# Autodesk Inventor assembly: CuboidSecurityBox
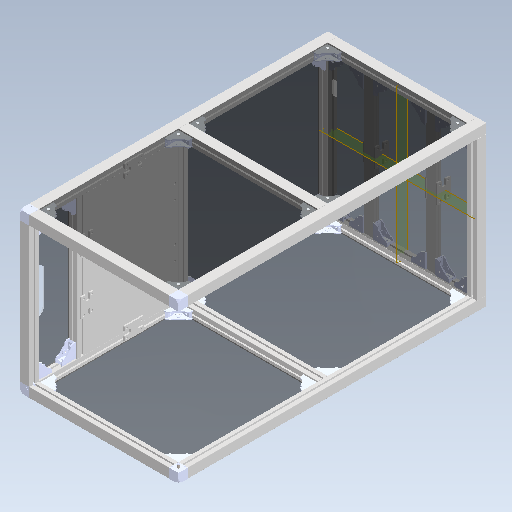
[picture p0: Inventor's stored thumbnail of the model, 512x512]
Saved by Autodesk Inventor 2021 (Build 250183000, 183)
## iProperties
Created: 2020-11-05
Part Number: CuboidSecurityBox
Document SubType Name: Assembly
Designer: gisen
Author: gisen
## Documents named in this file (12)
- D:\GitProjects\CAD-Data\CuboidAccessories\SecurityBox\Assemblies\CuboidSecurityBoxBasis.iam
- D:\GitProjects\CAD-Data\CuboidAccessories\SecurityBox\Frames\BasicFrameSingleSide290.ipt
- D:\GitProjects\CAD-Data\GeneralComponentsTemplate\Fittings\BasicFrameBracket.ipt
- D:\GitProjects\CAD-Data\CuboidAccessories\SecurityBox\Frames\BasicFrameCornerSide620.ipt
- D:\GitProjects\CAD-Data\CuboidAccessories\SecurityBox\Frames\BasicFrameLight290.ipt
- D:\GitProjects\CAD-Data\CuboidAccessories\SecurityBox\Misc\HTypeMount.ipt
- D:\GitProjects\CAD-Data\GeneralComponentsTemplate\Fittings\BasicFrameCubeBracket.iam
- D:\GitProjects\CAD-Data\CuboidAccessories\SecurityBox\Plates\InsideBottomPlate.ipt
- D:\GitProjects\CAD-Data\CuboidAccessories\SecurityBox\Assemblies\iPadHolderAssembly.iam
- D:\GitProjects\CAD-Data\CuboidAccessories\SecurityBox\Frames\BasicFrameCornerSide290.ipt
- D:\GitProjects\CAD-Data\CuboidAccessories\SecurityBox\Plates\OutsideSidePlate.ipt
- D:\GitProjects\CAD-Data\CuboidAccessories\SecurityBox\Plates\OutsideBackSideHigherPlate.ipt
## Components (73 placed, 11 different names)
1. BasicFrameSingleSide290:1 — フラッシュ:3, メイト:38, メイト:39, フラッシュ:21, フラッシュ:23, メイト:41, メイト:52, メイト:60, メイト:62, メイト:64, メイト:65, メイト:129, メイト:177, メイト:224, 対称度:1
2. BasicFrameSingleSide290:2 — フラッシュ:22, フラッシュ:24, フラッシュ:25, フラッシュ:26, メイト:40, メイト:42, メイト:43, メイト:44, メイト:45, メイト:104, メイト:107, メイト:110, メイト:113, フラッシュ:43, メイト:128, 対称度:2, メイト:239, メイト:241
3. BasicFrameSingleSide290:3 — フラッシュ:15, フラッシュ:18, メイト:35, フラッシュ:27, メイト:46, メイト:47, メイト:50, メイト:55, メイト:67, メイト:68, メイト:69, メイト:71, メイト:214, メイト:218, 対称度:1
4. BasicFrameSingleSide290:4 — フラッシュ:3, フラッシュ:16, フラッシュ:17, メイト:36, フラッシュ:19, メイト:37, フラッシュ:20, メイト:48, メイト:49, メイト:51, メイト:53, メイト:54, メイト:56, メイト:57, メイト:59, フラッシュ:32, フラッシュ:33, メイト:92, メイト:95, メイト:98, メイト:101, 対称度:2
5. BasicFrameBracket:23 — メイト:48, メイト:49, メイト:50
6. BasicFrameBracket:27 — メイト:45, メイト:46, メイト:47
7. BasicFrameBracket:28 — メイト:51, メイト:52, メイト:53
8. BasicFrameCornerSide620:1 — フラッシュ:25, フラッシュ:26, メイト:40, フラッシュ:27, メイト:66, メイト:126, フラッシュ:39, フラッシュ:40, メイト:158, メイト:157, メイト:183, メイト:203, メイト:204, メイト:215
9. BasicFrameCornerSide620:2 — メイト:39, フラッシュ:21, フラッシュ:22, フラッシュ:23, フラッシュ:24, メイト:43, メイト:63, メイト:127, フラッシュ:41, フラッシュ:42, メイト:167, メイト:168, メイト:169, メイト:191, フラッシュ:80, メイト:199, メイト:201, メイト:223
10. BasicFrameCornerSide620:3 — フラッシュ:19, メイト:37, フラッシュ:20, メイト:38, メイト:58, メイト:61, メイト:135, フラッシュ:47, メイト:147, フラッシュ:52, フラッシュ:53, メイト:163, メイト:165, フラッシュ:61, メイト:187, メイト:197, メイト:198, メイト:211, メイト:213, メイト:220, メイト:222
11. BasicFrameCornerSide620:4 — フラッシュ:15, フラッシュ:16, フラッシュ:17, フラッシュ:18, メイト:35, メイト:36, メイト:70, メイト:148, フラッシュ:54, フラッシュ:55, メイト:154, メイト:159, メイト:161, メイト:172, フラッシュ:63, メイト:186, メイト:205, メイト:207, メイト:209, メイト:210, メイト:217, メイト:226
12. BasicFrameBracket:29 — メイト:41, メイト:42, メイト:44
13. BasicFrameBracket:30 — メイト:54, メイト:55, メイト:56
14. BasicFrameBracket:31 — メイト:57, メイト:58, メイト:59
15. BasicFrameBracket:33 — メイト:66, メイト:67, メイト:68
16. BasicFrameBracket:34 — メイト:69, メイト:70, メイト:71
17. BasicFrameBracket:35 — メイト:63, メイト:64, メイト:65
18. BasicFrameBracket:37 — メイト:60, メイト:61, メイト:62
19. BasicFrameLight290:1 — フラッシュ:32, メイト:88, メイト:91, メイト:93, メイト:102, メイト:106, メイト:120, メイト:121, メイト:122, メイト:123, メイト:124, メイト:125, フラッシュ:64, フラッシュ:65, フラッシュ:66, フラッシュ:67, フラッシュ:68, メイト:177
20. BasicFrameLight290:2 — フラッシュ:33, メイト:88, メイト:97, メイト:99, メイト:108, メイト:112, メイト:114, メイト:115, メイト:116, メイト:117, メイト:118, メイト:119, フラッシュ:68, フラッシュ:69, フラッシュ:70, フラッシュ:71, フラッシュ:72, フラッシュ:73, メイト:241
21. BasicFrameBracket:38 — メイト:91, メイト:92, フラッシュ:64
22. BasicFrameBracket:39 — メイト:93, メイト:95, フラッシュ:65
23. BasicFrameBracket:40 — メイト:102, メイト:104, フラッシュ:66
24. BasicFrameBracket:41 — メイト:106, メイト:107, フラッシュ:67
25. BasicFrameBracket:42 — メイト:97, メイト:98, フラッシュ:69
26. BasicFrameBracket:43 — メイト:99, メイト:101, フラッシュ:70
27. BasicFrameBracket:44 — メイト:108, メイト:110, フラッシュ:71
28. BasicFrameBracket:45 — メイト:112, メイト:113, フラッシュ:72
29. HTypeMount:1 — メイト:114, メイト:115, メイト:116, フラッシュ:35
30. HTypeMount:2 — メイト:117, メイト:118, メイト:119, フラッシュ:35, フラッシュ:37, フラッシュ:73
31. HTypeMount:3 — メイト:123, メイト:124, メイト:125, フラッシュ:36, フラッシュ:37
32. HTypeMount:4 — メイト:120, メイト:121, メイト:122, フラッシュ:36
33. BasicFrameCubeBracket:1 [sub-assembly] — メイト:126, フラッシュ:39, フラッシュ:40, フラッシュ:76
34. BasicFrameCubeBracket:2 [sub-assembly] — メイト:127, フラッシュ:41, フラッシュ:42, メイト:195
35. InsideBottomPlate:1 — フラッシュ:43, メイト:128, メイト:129
36. BasicFrameSingleSide290:5 — メイト:130, メイト:131, フラッシュ:44, メイト:132, メイト:133, フラッシュ:45, メイト:134, フラッシュ:46, フラッシュ:47, フラッシュ:48, フラッシュ:57, フラッシュ:60, フラッシュ:62, フラッシュ:83, メイト:219
37. BasicFrameBracket:46 — メイト:130, メイト:131, フラッシュ:44, メイト:135
38. BasicFrameBracket:47 — メイト:132, メイト:133, フラッシュ:45
39. BasicFrameSingleSide290:6 — メイト:134, フラッシュ:46, フラッシュ:48, メイト:137, メイト:138, メイト:139, メイト:140, フラッシュ:50, フラッシュ:51, メイト:153, フラッシュ:88, メイト:225
40. BasicFrameBracket:48 — メイト:139, メイト:140, フラッシュ:50
41. BasicFrameBracket:49 — メイト:137, メイト:138, フラッシュ:51
42. BasicFrameCubeBracket:3 [sub-assembly] — メイト:147, フラッシュ:52, フラッシュ:53, メイト:194
43. BasicFrameCubeBracket:4 [sub-assembly] — メイト:148, フラッシュ:54, フラッシュ:55, メイト:193, フラッシュ:75, フラッシュ:77, フラッシュ:78
44. iPadHolderAssembly:1 [sub-assembly] — メイト:153, フラッシュ:57, メイト:154, メイト:227, メイト:228, メイト:229, メイト:230, メイト:231, メイト:232, メイト:233, メイト:234, メイト:235, メイト:236, メイト:237, メイト:238
45. BasicFrameBracket:52 — メイト:157, メイト:158, メイト:174
46. BasicFrameBracket:53 — メイト:163, メイト:165, メイト:171
47. BasicFrameBracket:54 — メイト:159, メイト:161, メイト:173
48. BasicFrameBracket:55 — メイト:167, メイト:168, メイト:170
49. BasicFrameSingleSide290:7 — メイト:169, メイト:170, フラッシュ:60, メイト:171, フラッシュ:61, メイト:188, メイト:189, メイト:190, メイト:192, フラッシュ:84, フラッシュ:85
50. BasicFrameSingleSide290:8 — メイト:172, フラッシュ:62, フラッシュ:63, メイト:173, メイト:174, メイト:181, メイト:182, メイト:184, メイト:185, メイト:214, フラッシュ:82
51. BasicFrameBracket:56 — メイト:181, メイト:182, メイト:183
52. BasicFrameBracket:57 — メイト:184, メイト:185, メイト:186
53. BasicFrameBracket:58 — メイト:187, メイト:188, メイト:189
54. BasicFrameBracket:59 — メイト:190, メイト:191, メイト:192
55. BasicFrameCornerSide290:1 — メイト:193, フラッシュ:75, フラッシュ:76, メイト:202, メイト:206, フラッシュ:81, メイト:216
56. BasicFrameCornerSide290:3 — メイト:194, フラッシュ:77, フラッシュ:78, フラッシュ:79, メイト:208, メイト:212
57. BasicFrameCornerSide290:4 — メイト:195, フラッシュ:79, フラッシュ:80, メイト:196, メイト:200, メイト:221
58. BasicFrameBracket:60 — メイト:196, メイト:197, メイト:198
59. BasicFrameBracket:61 — メイト:199, メイト:200, メイト:201
60. BasicFrameBracket:62 — メイト:202, メイト:203, メイト:204
61. BasicFrameBracket:63 — メイト:205, メイト:206, メイト:207
62. BasicFrameBracket:64 — メイト:211, メイト:212, メイト:213
63. BasicFrameBracket:65 — メイト:208, メイト:209, メイト:210
64. OutsideSidePlate:1 — フラッシュ:83, メイト:219, メイト:220
65. OutsideSidePlate:2 — フラッシュ:82, メイト:217, メイト:218
66. OutsideSidePlate:3 — フラッシュ:81, メイト:215, メイト:216
67. OutsideSidePlate:4 — フラッシュ:85, メイト:223, メイト:224
68. OutsideSidePlate:5 — フラッシュ:84, メイト:221, メイト:222
69. OutsideBackSideHigherPlate:1 — フラッシュ:88, メイト:225, メイト:226
70. HTypeMount:5 — メイト:236, メイト:237, メイト:238
71. HTypeMount:6 — メイト:233, メイト:234, メイト:235
72. HTypeMount:7 — メイト:227, メイト:228, メイト:229
73. HTypeMount:8 — メイト:230, メイト:231, メイト:232
## Relationships (225: Mate 161, Flush 62, Symmetry 2)
- フラッシュ:3 [Flush]: BasicFrameSingleSide290:1 ↔ BasicFrameSingleSide290:4
- フラッシュ:15 [Flush]: BasicFrameSingleSide290:3 ↔ BasicFrameCornerSide620:4
- フラッシュ:16 [Flush]: BasicFrameSingleSide290:4 ↔ BasicFrameCornerSide620:4
- フラッシュ:17 [Flush]: BasicFrameSingleSide290:4 ↔ BasicFrameCornerSide620:4
- フラッシュ:18 [Flush]: BasicFrameSingleSide290:3 ↔ BasicFrameCornerSide620:4
- メイト:35 [Mate]: BasicFrameSingleSide290:3 ↔ BasicFrameCornerSide620:4
- メイト:36 [Mate]: BasicFrameSingleSide290:4 ↔ BasicFrameCornerSide620:4
- フラッシュ:19 [Flush]: BasicFrameSingleSide290:4 ↔ BasicFrameCornerSide620:3
- メイト:37 [Mate]: BasicFrameSingleSide290:4 ↔ BasicFrameCornerSide620:3
- フラッシュ:20 [Flush]: BasicFrameSingleSide290:4 ↔ BasicFrameCornerSide620:3
- メイト:38 [Mate]: BasicFrameSingleSide290:1 ↔ BasicFrameCornerSide620:3
- メイト:39 [Mate]: BasicFrameSingleSide290:1 ↔ BasicFrameCornerSide620:2
- フラッシュ:21 [Flush]: BasicFrameSingleSide290:1 ↔ BasicFrameCornerSide620:2
- フラッシュ:22 [Flush]: BasicFrameSingleSide290:2 ↔ BasicFrameCornerSide620:2
- フラッシュ:23 [Flush]: BasicFrameSingleSide290:1 ↔ BasicFrameCornerSide620:2
- フラッシュ:24 [Flush]: BasicFrameSingleSide290:2 ↔ BasicFrameCornerSide620:2
- フラッシュ:25 [Flush]: BasicFrameSingleSide290:2 ↔ BasicFrameCornerSide620:1
- フラッシュ:26 [Flush]: BasicFrameSingleSide290:2 ↔ BasicFrameCornerSide620:1
- メイト:40 [Mate]: BasicFrameSingleSide290:2 ↔ BasicFrameCornerSide620:1
- メイト:41 [Mate]: BasicFrameSingleSide290:1 ↔ BasicFrameBracket:29
- メイト:42 [Mate] (-10 mm): BasicFrameSingleSide290:2 ↔ BasicFrameBracket:29
- メイト:43 [Mate]: BasicFrameSingleSide290:2 ↔ BasicFrameCornerSide620:2
- フラッシュ:27 [Flush]: BasicFrameSingleSide290:3 ↔ BasicFrameCornerSide620:1
- メイト:44 [Mate]: BasicFrameSingleSide290:2 ↔ BasicFrameBracket:29
- メイト:45 [Mate]: BasicFrameSingleSide290:2 ↔ BasicFrameBracket:27
- メイト:46 [Mate]: BasicFrameSingleSide290:3 ↔ BasicFrameBracket:27
- メイト:47 [Mate] (-10 mm): BasicFrameSingleSide290:3 ↔ BasicFrameBracket:27
- メイト:48 [Mate]: BasicFrameSingleSide290:4 ↔ BasicFrameBracket:23
- メイト:49 [Mate] (-10 mm): BasicFrameSingleSide290:4 ↔ BasicFrameBracket:23
- メイト:50 [Mate]: BasicFrameSingleSide290:3 ↔ BasicFrameBracket:23
- メイト:51 [Mate]: BasicFrameSingleSide290:4 ↔ BasicFrameBracket:28
- メイト:52 [Mate]: BasicFrameSingleSide290:1 ↔ BasicFrameBracket:28
- メイト:53 [Mate] (-10 mm): BasicFrameSingleSide290:4 ↔ BasicFrameBracket:28
- メイト:54 [Mate]: BasicFrameSingleSide290:4 ↔ BasicFrameBracket:30
- メイト:55 [Mate]: BasicFrameSingleSide290:3 ↔ BasicFrameBracket:30
- メイト:56 [Mate] (-10 mm): BasicFrameSingleSide290:4 ↔ BasicFrameBracket:30
- メイト:57 [Mate]: BasicFrameSingleSide290:4 ↔ BasicFrameBracket:31
- メイト:58 [Mate]: BasicFrameCornerSide620:3 ↔ BasicFrameBracket:31
- メイト:59 [Mate] (-10 mm): BasicFrameSingleSide290:4 ↔ BasicFrameBracket:31
- メイト:60 [Mate] (-10 mm): BasicFrameSingleSide290:1 ↔ BasicFrameBracket:37
- メイト:61 [Mate]: BasicFrameCornerSide620:3 ↔ BasicFrameBracket:37
- メイト:62 [Mate]: BasicFrameSingleSide290:1 ↔ BasicFrameBracket:37
- メイト:63 [Mate]: BasicFrameCornerSide620:2 ↔ BasicFrameBracket:35
- メイト:64 [Mate]: BasicFrameSingleSide290:1 ↔ BasicFrameBracket:35
- メイト:65 [Mate] (-10 mm): BasicFrameSingleSide290:1 ↔ BasicFrameBracket:35
- メイト:66 [Mate]: BasicFrameCornerSide620:1 ↔ BasicFrameBracket:33
- メイト:67 [Mate]: BasicFrameSingleSide290:3 ↔ BasicFrameBracket:33
- メイト:68 [Mate] (-10 mm): BasicFrameSingleSide290:3 ↔ BasicFrameBracket:33
- メイト:69 [Mate]: BasicFrameSingleSide290:3 ↔ BasicFrameBracket:34
- メイト:70 [Mate]: BasicFrameCornerSide620:4 ↔ BasicFrameBracket:34
- メイト:71 [Mate] (-10 mm): BasicFrameSingleSide290:3 ↔ BasicFrameBracket:34
- フラッシュ:32 [Flush] (5 mm): BasicFrameSingleSide290:4 ↔ BasicFrameLight290:1
- フラッシュ:33 [Flush] (5 mm): BasicFrameSingleSide290:4 ↔ BasicFrameLight290:2
- メイト:88 [Mate] (110 mm): BasicFrameLight290:1 ↔ BasicFrameLight290:2
- メイト:91 [Mate]: BasicFrameLight290:1 ↔ BasicFrameBracket:38
- メイト:92 [Mate] (-10 mm): BasicFrameSingleSide290:4 ↔ BasicFrameBracket:38
- メイト:93 [Mate]: BasicFrameLight290:1 ↔ BasicFrameBracket:39
- メイト:95 [Mate] (-10 mm): BasicFrameSingleSide290:4 ↔ BasicFrameBracket:39
- メイト:97 [Mate]: BasicFrameLight290:2 ↔ BasicFrameBracket:42
- メイト:98 [Mate] (-10 mm): BasicFrameSingleSide290:4 ↔ BasicFrameBracket:42
- メイト:99 [Mate]: BasicFrameLight290:2 ↔ BasicFrameBracket:43
- メイト:101 [Mate] (-10 mm): BasicFrameSingleSide290:4 ↔ BasicFrameBracket:43
- メイト:102 [Mate]: BasicFrameLight290:1 ↔ BasicFrameBracket:40
- メイト:104 [Mate] (-10 mm): BasicFrameSingleSide290:2 ↔ BasicFrameBracket:40
- メイト:106 [Mate]: BasicFrameLight290:1 ↔ BasicFrameBracket:41
- メイト:107 [Mate] (-10 mm): BasicFrameSingleSide290:2 ↔ BasicFrameBracket:41
- メイト:108 [Mate]: BasicFrameLight290:2 ↔ BasicFrameBracket:44
- メイト:110 [Mate] (-10 mm): BasicFrameSingleSide290:2 ↔ BasicFrameBracket:44
- メイト:112 [Mate]: BasicFrameLight290:2 ↔ BasicFrameBracket:45
- メイト:113 [Mate] (-10 mm): BasicFrameSingleSide290:2 ↔ BasicFrameBracket:45
- メイト:114 [Mate]: BasicFrameLight290:2 ↔ HTypeMount:1
- メイト:115 [Mate] (-5 mm): BasicFrameLight290:2 ↔ HTypeMount:1
- メイト:116 [Mate] (-5 mm): BasicFrameLight290:2 ↔ HTypeMount:1
- メイト:117 [Mate]: BasicFrameLight290:2 ↔ HTypeMount:2
- メイト:118 [Mate] (-5 mm): BasicFrameLight290:2 ↔ HTypeMount:2
- メイト:119 [Mate] (-5 mm): BasicFrameLight290:2 ↔ HTypeMount:2
- フラッシュ:35 [Flush]: HTypeMount:1 ↔ HTypeMount:2
- メイト:120 [Mate]: BasicFrameLight290:1 ↔ HTypeMount:4
- メイト:121 [Mate] (-5 mm): BasicFrameLight290:1 ↔ HTypeMount:4
- メイト:122 [Mate] (-5 mm): BasicFrameLight290:1 ↔ HTypeMount:4
- メイト:123 [Mate]: BasicFrameLight290:1 ↔ HTypeMount:3
- メイト:124 [Mate] (-5 mm): BasicFrameLight290:1 ↔ HTypeMount:3
- メイト:125 [Mate] (-5 mm): BasicFrameLight290:1 ↔ HTypeMount:3
- フラッシュ:36 [Flush]: HTypeMount:3 ↔ HTypeMount:4
- フラッシュ:37 [Flush]: HTypeMount:2 ↔ HTypeMount:3
- メイト:126 [Mate]: BasicFrameCornerSide620:1 ↔ BasicFrameCubeBracket:1
- フラッシュ:39 [Flush]: BasicFrameCornerSide620:1 ↔ BasicFrameCubeBracket:1
- フラッシュ:40 [Flush]: BasicFrameCornerSide620:1 ↔ BasicFrameCubeBracket:1
- メイト:127 [Mate]: BasicFrameCornerSide620:2 ↔ BasicFrameCubeBracket:2
- フラッシュ:41 [Flush]: BasicFrameCornerSide620:2 ↔ BasicFrameCubeBracket:2
- フラッシュ:42 [Flush]: BasicFrameCornerSide620:2 ↔ BasicFrameCubeBracket:2
- フラッシュ:43 [Flush]: BasicFrameSingleSide290:2 ↔ InsideBottomPlate:1
- メイト:128 [Mate]: BasicFrameSingleSide290:2 ↔ InsideBottomPlate:1
- メイト:129 [Mate]: BasicFrameSingleSide290:1 ↔ InsideBottomPlate:1
- メイト:130 [Mate]: BasicFrameSingleSide290:5 ↔ BasicFrameBracket:46
- メイト:131 [Mate] (-10 mm): BasicFrameSingleSide290:5 ↔ BasicFrameBracket:46
- フラッシュ:44 [Flush]: BasicFrameSingleSide290:5 ↔ BasicFrameBracket:46
- メイト:132 [Mate]: BasicFrameSingleSide290:5 ↔ BasicFrameBracket:47
- メイト:133 [Mate] (-10 mm): BasicFrameSingleSide290:5 ↔ BasicFrameBracket:47
- フラッシュ:45 [Flush]: BasicFrameSingleSide290:5 ↔ BasicFrameBracket:47
- メイト:134 [Mate] (190 mm): BasicFrameSingleSide290:5 ↔ BasicFrameSingleSide290:6
- フラッシュ:46 [Flush]: BasicFrameSingleSide290:5 ↔ BasicFrameSingleSide290:6
- メイト:135 [Mate]: BasicFrameCornerSide620:3 ↔ BasicFrameBracket:46
- フラッシュ:47 [Flush]: BasicFrameCornerSide620:3 ↔ BasicFrameSingleSide290:5
- フラッシュ:48 [Flush]: BasicFrameSingleSide290:5 ↔ BasicFrameSingleSide290:6
- メイト:137 [Mate]: BasicFrameSingleSide290:6 ↔ BasicFrameBracket:49
- メイト:138 [Mate] (-10 mm): BasicFrameSingleSide290:6 ↔ BasicFrameBracket:49
- メイト:139 [Mate]: BasicFrameSingleSide290:6 ↔ BasicFrameBracket:48
- メイト:140 [Mate] (-10 mm): BasicFrameSingleSide290:6 ↔ BasicFrameBracket:48
- フラッシュ:50 [Flush]: BasicFrameSingleSide290:6 ↔ BasicFrameBracket:48
- フラッシュ:51 [Flush]: BasicFrameSingleSide290:6 ↔ BasicFrameBracket:49
- メイト:147 [Mate]: BasicFrameCornerSide620:3 ↔ BasicFrameCubeBracket:3
- フラッシュ:52 [Flush]: BasicFrameCornerSide620:3 ↔ BasicFrameCubeBracket:3
- フラッシュ:53 [Flush]: BasicFrameCornerSide620:3 ↔ BasicFrameCubeBracket:3
- メイト:148 [Mate]: BasicFrameCornerSide620:4 ↔ BasicFrameCubeBracket:4
- フラッシュ:54 [Flush]: BasicFrameCornerSide620:4 ↔ BasicFrameCubeBracket:4
- フラッシュ:55 [Flush]: BasicFrameCornerSide620:4 ↔ BasicFrameCubeBracket:4
- メイト:153 [Mate]: BasicFrameSingleSide290:6 ↔ iPadHolderAssembly:1
- フラッシュ:57 [Flush]: BasicFrameSingleSide290:5 ↔ iPadHolderAssembly:1
- メイト:154 [Mate]: BasicFrameCornerSide620:4 ↔ iPadHolderAssembly:1
- メイト:157 [Mate] (-10 mm): BasicFrameCornerSide620:1 ↔ BasicFrameBracket:52
- メイト:158 [Mate]: BasicFrameCornerSide620:1 ↔ BasicFrameBracket:52
- メイト:159 [Mate]: BasicFrameCornerSide620:4 ↔ BasicFrameBracket:54
- メイト:161 [Mate] (-10 mm): BasicFrameCornerSide620:4 ↔ BasicFrameBracket:54
- メイト:163 [Mate]: BasicFrameCornerSide620:3 ↔ BasicFrameBracket:53
- メイト:165 [Mate] (-10 mm): BasicFrameCornerSide620:3 ↔ BasicFrameBracket:53
- メイト:167 [Mate]: BasicFrameCornerSide620:2 ↔ BasicFrameBracket:55
- メイト:168 [Mate] (-10 mm): BasicFrameCornerSide620:2 ↔ BasicFrameBracket:55
- メイト:169 [Mate]: BasicFrameCornerSide620:2 ↔ BasicFrameSingleSide290:7
- メイト:170 [Mate]: BasicFrameBracket:55 ↔ BasicFrameSingleSide290:7
- フラッシュ:60 [Flush]: BasicFrameSingleSide290:5 ↔ BasicFrameSingleSide290:7
- メイト:171 [Mate]: BasicFrameBracket:53 ↔ BasicFrameSingleSide290:7
- フラッシュ:61 [Flush]: BasicFrameCornerSide620:3 ↔ BasicFrameSingleSide290:7
- メイト:172 [Mate]: BasicFrameCornerSide620:4 ↔ BasicFrameSingleSide290:8
- フラッシュ:62 [Flush]: BasicFrameSingleSide290:5 ↔ BasicFrameSingleSide290:8
- フラッシュ:63 [Flush]: BasicFrameCornerSide620:4 ↔ BasicFrameSingleSide290:8
- メイト:173 [Mate]: BasicFrameBracket:54 ↔ BasicFrameSingleSide290:8
- メイト:174 [Mate]: BasicFrameBracket:52 ↔ BasicFrameSingleSide290:8
- フラッシュ:64 [Flush]: BasicFrameLight290:1 ↔ BasicFrameBracket:38
- フラッシュ:65 [Flush]: BasicFrameLight290:1 ↔ BasicFrameBracket:39
- フラッシュ:66 [Flush]: BasicFrameLight290:1 ↔ BasicFrameBracket:40
- フラッシュ:67 [Flush]: BasicFrameLight290:1 ↔ BasicFrameBracket:41
- フラッシュ:68 [Flush]: BasicFrameLight290:1 ↔ BasicFrameLight290:2
- フラッシュ:69 [Flush]: BasicFrameLight290:2 ↔ BasicFrameBracket:42
- フラッシュ:70 [Flush]: BasicFrameLight290:2 ↔ BasicFrameBracket:43
- フラッシュ:71 [Flush]: BasicFrameLight290:2 ↔ BasicFrameBracket:44
- フラッシュ:72 [Flush]: BasicFrameLight290:2 ↔ BasicFrameBracket:45
- フラッシュ:73 [Flush] (-125 mm): BasicFrameLight290:2 ↔ HTypeMount:2
- メイト:177 [Mate]: BasicFrameSingleSide290:1 ↔ BasicFrameLight290:1
- メイト:181 [Mate]: BasicFrameSingleSide290:8 ↔ BasicFrameBracket:56
- メイト:182 [Mate] (-10 mm): BasicFrameSingleSide290:8 ↔ BasicFrameBracket:56
- メイト:183 [Mate]: BasicFrameCornerSide620:1 ↔ BasicFrameBracket:56
- メイト:184 [Mate]: BasicFrameSingleSide290:8 ↔ BasicFrameBracket:57
- メイト:185 [Mate] (-10 mm): BasicFrameSingleSide290:8 ↔ BasicFrameBracket:57
- メイト:186 [Mate]: BasicFrameCornerSide620:4 ↔ BasicFrameBracket:57
- メイト:187 [Mate]: BasicFrameCornerSide620:3 ↔ BasicFrameBracket:58
- メイト:188 [Mate]: BasicFrameSingleSide290:7 ↔ BasicFrameBracket:58
- メイト:189 [Mate] (-10 mm): BasicFrameSingleSide290:7 ↔ BasicFrameBracket:58
- メイト:190 [Mate]: BasicFrameSingleSide290:7 ↔ BasicFrameBracket:59
- メイト:191 [Mate]: BasicFrameCornerSide620:2 ↔ BasicFrameBracket:59
- メイト:192 [Mate] (-10 mm): BasicFrameSingleSide290:7 ↔ BasicFrameBracket:59
- メイト:193 [Mate]: BasicFrameCubeBracket:4 ↔ BasicFrameCornerSide290:1
- フラッシュ:75 [Flush]: BasicFrameCubeBracket:4 ↔ BasicFrameCornerSide290:1
- フラッシュ:76 [Flush]: BasicFrameCubeBracket:1 ↔ BasicFrameCornerSide290:1
- メイト:194 [Mate]: BasicFrameCubeBracket:3 ↔ BasicFrameCornerSide290:3
- フラッシュ:77 [Flush]: BasicFrameCubeBracket:4 ↔ BasicFrameCornerSide290:3
- フラッシュ:78 [Flush]: BasicFrameCubeBracket:4 ↔ BasicFrameCornerSide290:3
- メイト:195 [Mate]: BasicFrameCubeBracket:2 ↔ BasicFrameCornerSide290:4
- フラッシュ:79 [Flush]: BasicFrameCornerSide290:3 ↔ BasicFrameCornerSide290:4
- フラッシュ:80 [Flush]: BasicFrameCornerSide620:2 ↔ BasicFrameCornerSide290:4
- メイト:196 [Mate]: BasicFrameCornerSide290:4 ↔ BasicFrameBracket:60
- メイト:197 [Mate]: BasicFrameCornerSide620:3 ↔ BasicFrameBracket:60
- メイト:198 [Mate] (-10 mm): BasicFrameCornerSide620:3 ↔ BasicFrameBracket:60
- メイト:199 [Mate]: BasicFrameCornerSide620:2 ↔ BasicFrameBracket:61
- メイト:200 [Mate]: BasicFrameCornerSide290:4 ↔ BasicFrameBracket:61
- メイト:201 [Mate] (-10 mm): BasicFrameCornerSide620:2 ↔ BasicFrameBracket:61
- メイト:202 [Mate]: BasicFrameCornerSide290:1 ↔ BasicFrameBracket:62
- メイト:203 [Mate]: BasicFrameCornerSide620:1 ↔ BasicFrameBracket:62
- メイト:204 [Mate] (-10 mm): BasicFrameCornerSide620:1 ↔ BasicFrameBracket:62
- メイト:205 [Mate]: BasicFrameCornerSide620:4 ↔ BasicFrameBracket:63
- メイト:206 [Mate]: BasicFrameCornerSide290:1 ↔ BasicFrameBracket:63
- メイト:207 [Mate] (-10 mm): BasicFrameCornerSide620:4 ↔ BasicFrameBracket:63
- メイト:208 [Mate]: BasicFrameCornerSide290:3 ↔ BasicFrameBracket:65
- メイト:209 [Mate]: BasicFrameCornerSide620:4 ↔ BasicFrameBracket:65
- メイト:210 [Mate] (-10 mm): BasicFrameCornerSide620:4 ↔ BasicFrameBracket:65
- メイト:211 [Mate]: BasicFrameCornerSide620:3 ↔ BasicFrameBracket:64
- メイト:212 [Mate]: BasicFrameCornerSide290:3 ↔ BasicFrameBracket:64
- メイト:213 [Mate] (-10 mm): BasicFrameCornerSide620:3 ↔ BasicFrameBracket:64
- メイト:214 [Mate] (290 mm): BasicFrameSingleSide290:3 ↔ BasicFrameSingleSide290:8
- フラッシュ:81 [Flush]: BasicFrameCornerSide290:1 ↔ OutsideSidePlate:3
- メイト:215 [Mate]: BasicFrameCornerSide620:1 ↔ OutsideSidePlate:3
- メイト:216 [Mate]: BasicFrameCornerSide290:1 ↔ OutsideSidePlate:3
- フラッシュ:82 [Flush]: BasicFrameSingleSide290:8 ↔ OutsideSidePlate:2
- メイト:217 [Mate]: BasicFrameCornerSide620:4 ↔ OutsideSidePlate:2
- メイト:218 [Mate]: BasicFrameSingleSide290:3 ↔ OutsideSidePlate:2
- フラッシュ:83 [Flush]: BasicFrameSingleSide290:5 ↔ OutsideSidePlate:1
- メイト:219 [Mate]: BasicFrameSingleSide290:5 ↔ OutsideSidePlate:1
- メイト:220 [Mate]: BasicFrameCornerSide620:3 ↔ OutsideSidePlate:1
- フラッシュ:84 [Flush]: BasicFrameSingleSide290:7 ↔ OutsideSidePlate:5
- メイト:221 [Mate]: BasicFrameCornerSide290:4 ↔ OutsideSidePlate:5
- メイト:222 [Mate]: BasicFrameCornerSide620:3 ↔ OutsideSidePlate:5
- フラッシュ:85 [Flush]: BasicFrameSingleSide290:7 ↔ OutsideSidePlate:4
- メイト:223 [Mate]: BasicFrameCornerSide620:2 ↔ OutsideSidePlate:4
- メイト:224 [Mate]: BasicFrameSingleSide290:1 ↔ OutsideSidePlate:4
- フラッシュ:88 [Flush]: BasicFrameSingleSide290:6 ↔ OutsideBackSideHigherPlate:1
- メイト:225 [Mate]: BasicFrameSingleSide290:6 ↔ OutsideBackSideHigherPlate:1
- メイト:226 [Mate]: BasicFrameCornerSide620:4 ↔ OutsideBackSideHigherPlate:1
- メイト:227 [Mate]: iPadHolderAssembly:1 ↔ HTypeMount:7
- メイト:228 [Mate]: iPadHolderAssembly:1 ↔ HTypeMount:7
- メイト:229 [Mate]: iPadHolderAssembly:1 ↔ HTypeMount:7
- メイト:230 [Mate]: iPadHolderAssembly:1 ↔ HTypeMount:8
- メイト:231 [Mate]: iPadHolderAssembly:1 ↔ HTypeMount:8
- メイト:232 [Mate]: iPadHolderAssembly:1 ↔ HTypeMount:8
- メイト:233 [Mate]: iPadHolderAssembly:1 ↔ HTypeMount:6
- メイト:234 [Mate]: iPadHolderAssembly:1 ↔ HTypeMount:6
- メイト:235 [Mate]: iPadHolderAssembly:1 ↔ HTypeMount:6
- メイト:236 [Mate]: iPadHolderAssembly:1 ↔ HTypeMount:5
- メイト:237 [Mate]: iPadHolderAssembly:1 ↔ HTypeMount:5
- メイト:238 [Mate]: iPadHolderAssembly:1 ↔ HTypeMount:5
- 対称度:1 [Symmetry]: BasicFrameSingleSide290:1 ↔ BasicFrameSingleSide290:3
- 対称度:2 [Symmetry]: BasicFrameSingleSide290:2 ↔ BasicFrameSingleSide290:4
- メイト:239 [Mate]: BasicFrameSingleSide290:2
- メイト:240 [Mate]
- メイト:241 [Mate] (70 mm): BasicFrameSingleSide290:2 ↔ BasicFrameLight290:2
- メイト:242 [Mate]
